# Autodesk Inventor assembly: Rear Crossbrace
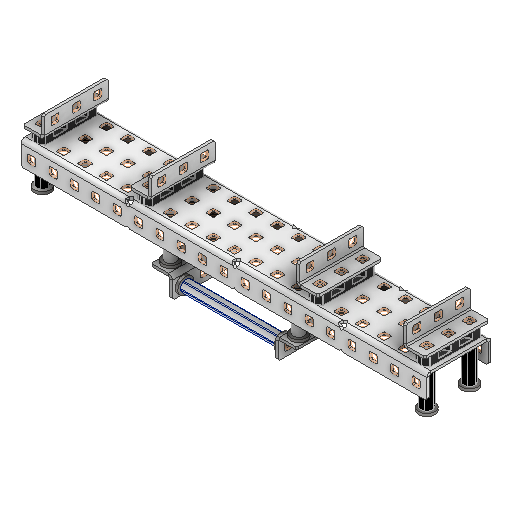
[picture p0: Inventor's stored thumbnail of the model, 512x512]
Saved by Autodesk Inventor 2025 (Build 290162000, 162)
## iProperties
Created: 2025-02-13
Part Number: Rear Crossbrace
Document SubType Name: Assembly
Designer: Averey Ku
Author: Averey Ku
## Documents named in this file (14)
- D:\VEX\High Stakes\CAD\V5\Chassis\Rear Crossbrace.iam
- D:\VEX\High Stakes\CAD\ROBOPROS-CAD-Inventor\Structure\C Channel\Aluminum 1x3x1\Alu C 1x3x1x19.ipt
- D:\VEX\High Stakes\CAD\ROBOPROS-CAD-Inventor\Structure\Angle\Aluminum 1x1\Alu Angle 1x1x3.ipt
- D:\VEX\High Stakes\CAD\ROBOPROS-CAD-Inventor\Motion\Shaft LS\Bearing Flat Low Profile.ipt
- D:\VEX\High Stakes\CAD\ROBOPROS-CAD-Inventor\Structure\Standoff\Standoff .875.ipt
- D:\VEX\High Stakes\CAD\ROBOPROS-CAD-Inventor\Structure\Standoff.ipt
- D:\VEX\High Stakes\CAD\ROBOPROS-CAD-Inventor\Motion\Spacers\Washer Steel\SWasher .375 OD x .062500.ipt
- D:\VEX\High Stakes\CAD\ROBOPROS-CAD-Inventor\Motion\Spacers\Washer Steel.ipt
- D:\VEX\High Stakes\CAD\ROBOPROS-CAD-Inventor\Motion\Spacers\Spacer Nylon .375 OD\NSpacer .375 OD x .125.ipt
- D:\VEX\High Stakes\CAD\ROBOPROS-CAD-Inventor\Motion\Spacers\Spacer Nylon .375 OD.ipt
- D:\VEX\High Stakes\CAD\ROBOPROS-CAD-Inventor\Motion\Spacers\Spacer Nylon .375 OD\NSpacer .375 OD x .500.ipt
- D:\VEX\High Stakes\CAD\ROBOPROS-CAD-Inventor\Structure\Nylon Standoff Rounded\Nylon Standoff .625.ipt
- D:\VEX\High Stakes\CAD\ROBOPROS-CAD-Inventor\Structure\Standoff\Standoff 2.25.ipt
- D:\VEX\High Stakes\CAD\ROBOPROS-CAD-Inventor\Motion\Spacers\Washer Steel\SWasher .375 OD x .031250.ipt
## Components (35 placed, 10 different names)
1. Alu C 1x3x1x19:1 — Flush:1, Insert:12, Insert:13, Insert:14, Insert:15, Flush:2, Flush:3, Insert:18, Mate:8, Insert:26, Mate:10, Insert:36, Mate:12, Insert:38, Mate:14
2. Alu Angle 1x1x3:1 — Insert:20, Mate:9
3. Alu Angle 1x1x3:2 — Insert:27, Insert:28, Insert:34
4. Bearing Flat Low Profile:1
5. Alu Angle 1x1x3:3
6. Alu Angle 1x1x3:4
7. Bearing Flat Low Profile:2
8. Standoff .875:4 — Insert:8, Insert:12
9. SWasher .375 OD x .062500:1 — Insert:8
10. Standoff .875:5 — Insert:13
11. SWasher .375 OD x .062500:2
12. Standoff .875:6 — Insert:14
13. SWasher .375 OD x .062500:3
14. Standoff .875:7 — Insert:15
15. SWasher .375 OD x .062500:4
16. Bearing Flat Low Profile:3 — Insert:18, Mate:8, Insert:21, Insert:22
17. NSpacer .375 OD x .125:1 — Insert:19, Insert:20, Insert:29
18. NSpacer .375 OD x .500:2 — Insert:19, Insert:21
19. Nylon Standoff .625:1 — Insert:22, Mate:9, Insert:30
20. Bearing Flat Low Profile:4 — Insert:26
21. NSpacer .375 OD x .125:5
22. NSpacer .375 OD x .500:6
23. Nylon Standoff .625:2 — Mate:10
24. SWasher .375 OD x .062500:5 — Insert:28
25. SWasher .375 OD x .062500:6 — Insert:27
26. SWasher .375 OD x .062500:7 — Insert:29
27. SWasher .375 OD x .062500:8 — Insert:30
28. Standoff 2.25:1 — Insert:31, Insert:32
29. SWasher .375 OD x .031250:9 — Insert:33
30. SWasher .375 OD x .062500:10 — Insert:32, Insert:33
31. SWasher .375 OD x .062500:11 — Insert:31, Insert:34
32. Alu Angle 1x1x3:5 — Mate:12
33. Bearing Flat Low Profile:5 — Insert:36
34. Alu Angle 1x1x3:6 — Mate:14
35. Bearing Flat Low Profile:6 — Insert:38
## Relationships (51: Insert 34, Mate 14, Flush 3)
- [Mate]: Alu C 1x3x1x19:1 ↔ Alu Angle 1x1x3:1
- [Mate]: Alu C 1x3x1x19:1 ↔ Alu Angle 1x1x3:1
- [Insert] (23.8125 mm): Alu C 1x3x1x19:1 ↔ Alu Angle 1x1x3:2
- [Mate]: Alu C 1x3x1x19:1 ↔ Alu Angle 1x1x3:2
- [Insert] (1.27 mm): Bearing Flat Low Profile:1 ↔ Alu Angle 1x1x3:3
- [Mate]: Bearing Flat Low Profile:1 ↔ Alu Angle 1x1x3:3
- [Insert]: Alu C 1x3x1x19:1 ↔ Bearing Flat Low Profile:2
- [Mate]: Alu C 1x3x1x19:1 ↔ Bearing Flat Low Profile:2
- [Insert] (1.27 mm): Alu Angle 1x1x3:4 ↔ Bearing Flat Low Profile:2
- [Mate]: Alu Angle 1x1x3:4 ↔ Bearing Flat Low Profile:2
- [Insert]: Alu C 1x3x1x19:1 ↔ Bearing Flat Low Profile:1
- [Mate]: Alu C 1x3x1x19:1 ↔ Alu Angle 1x1x3:3
- Flush:1 (-120.65 mm): Alu C 1x3x1x19:1
- Insert:8: Standoff .875:4 ↔ SWasher .375 OD x .062500:1
- [Insert]: Standoff .875:5 ↔ SWasher .375 OD x .062500:2
- [Insert]: Standoff .875:6 ↔ SWasher .375 OD x .062500:3
- [Insert]: Standoff .875:7 ↔ SWasher .375 OD x .062500:4
- Insert:12: Alu C 1x3x1x19:1 ↔ Standoff .875:4
- Insert:13: Alu C 1x3x1x19:1 ↔ Standoff .875:5
- Insert:14: Alu C 1x3x1x19:1 ↔ Standoff .875:6
- Insert:15: Alu C 1x3x1x19:1 ↔ Standoff .875:7
- Flush:2: Alu C 1x3x1x19:1
- Flush:3 (-19.05 mm): Alu C 1x3x1x19:1
- Insert:18: Alu C 1x3x1x19:1 ↔ Bearing Flat Low Profile:3
- Mate:8: Alu C 1x3x1x19:1 ↔ Bearing Flat Low Profile:3
- Insert:19: NSpacer .375 OD x .125:1 ↔ NSpacer .375 OD x .500:2
- Insert:20 (1.5875 mm): Alu Angle 1x1x3:1 ↔ NSpacer .375 OD x .125:1
- Insert:21 (1.27 mm): Bearing Flat Low Profile:3 ↔ NSpacer .375 OD x .500:2
- Insert:22 (1.27 mm): Bearing Flat Low Profile:3 ↔ Nylon Standoff .625:1
- Mate:9: Alu Angle 1x1x3:1 ↔ Nylon Standoff .625:1
- [Insert]: NSpacer .375 OD x .125:5 ↔ NSpacer .375 OD x .500:6
- [Insert] (1.27 mm): Bearing Flat Low Profile:4 ↔ NSpacer .375 OD x .500:6
- [Insert] (1.27 mm): Bearing Flat Low Profile:4 ↔ Nylon Standoff .625:2
- Insert:26: Alu C 1x3x1x19:1 ↔ Bearing Flat Low Profile:4
- Mate:10: Alu C 1x3x1x19:1 ↔ Nylon Standoff .625:2
- Insert:27: Alu Angle 1x1x3:2 ↔ SWasher .375 OD x .062500:6
- Insert:28: Alu Angle 1x1x3:2 ↔ SWasher .375 OD x .062500:5
- Insert:29: NSpacer .375 OD x .125:1 ↔ SWasher .375 OD x .062500:7
- Insert:30: Nylon Standoff .625:1 ↔ SWasher .375 OD x .062500:8
- Insert:31: Standoff 2.25:1 ↔ SWasher .375 OD x .062500:11
- Insert:32: Standoff 2.25:1 ↔ SWasher .375 OD x .062500:10
- Insert:33: SWasher .375 OD x .031250:9 ↔ SWasher .375 OD x .062500:10
- Insert:34: Alu Angle 1x1x3:2 ↔ SWasher .375 OD x .062500:11
- [Insert] (1.27 mm): Alu Angle 1x1x3:5 ↔ Bearing Flat Low Profile:5
- [Mate]: Alu Angle 1x1x3:5 ↔ Bearing Flat Low Profile:5
- Insert:36: Alu C 1x3x1x19:1 ↔ Bearing Flat Low Profile:5
- Mate:12: Alu C 1x3x1x19:1 ↔ Alu Angle 1x1x3:5
- [Insert] (1.27 mm): Alu Angle 1x1x3:6 ↔ Bearing Flat Low Profile:6
- [Mate]: Alu Angle 1x1x3:6 ↔ Bearing Flat Low Profile:6
- Insert:38: Alu C 1x3x1x19:1 ↔ Bearing Flat Low Profile:6
- Mate:14: Alu C 1x3x1x19:1 ↔ Alu Angle 1x1x3:6
## Named parameters: d220_d215 = 1.27 mm, d221_d216 = 0 mm, d16_d15 = 0 mm, d17_d15 = 0 mm, d18_d15 = 0 mm, d34_d29 = 0 mm, d35_d31 = 1.27 mm, d36_d32 = 1.27 mm, d60_d231 = 0 mm, d61_d230 = 1.27 mm, d64_d60_d231 = 0 mm, d65_d61_d230 = 1.27 mm
